# Autodesk Inventor assembly: main
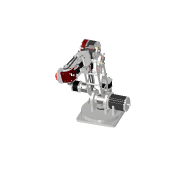
[picture p0: Inventor's stored thumbnail of the model, 180x180]
Saved by Autodesk Inventor 2020.3 (Build 243373000, 373)
## iProperties
Created: 2020-05-24
Part Number: main
Document SubType Name: Assembly
Designer: Svend
Author: Svend
## Documents named in this file (5)
- C:\Users\Svend\OneDrive\Documents\GitHub\BeerMinder\3D-model\mainAssembly\main.iam
- C:\Users\Svend\OneDrive\Documents\GitHub\BeerMinder\3D-model\axis3\axis3.iam
- C:\Users\Svend\OneDrive\Documents\GitHub\BeerMinder\3D-model\Base (Axis 1)\gefreesd\AssemblyGefreesdBasev2.iam
- C:\Users\Svend\OneDrive\Documents\GitHub\BeerMinder\3D-model\axis5_6\axis5_6  compact.iam
- C:\Users\Svend\OneDrive\Documents\GitHub\BeerMinder\3D-model\ControlBox\swithces\Assembly - V-156-1C25 micro switch (Idle).iam
## Components (8 placed, 4 different names)
1. axis3:1 [sub-assembly] — Mate:3, Mate:4, Mate:12, Mate:13, Mate:17, Mate:20, Mate:21, Mate:22, Mate:23, Mate:24, Mate:25, Mate:26, Mate:27
2. AssemblyGefreesdBasev2:1 [sub-assembly] — Mate:1, Mate:2, Flush:1, Mate:3, Mate:4, Mate:9, Mate:10, Angle:2, Flush:3
3. axis5_6  compact:1 [sub-assembly] — Mate:12, Mate:13
4. Assembly - V-156-1C25 micro switch (Idle):2 [sub-assembly]
5. Assembly - V-156-1C25 micro switch (Idle):1 [sub-assembly] — Mate:9, Mate:10, Angle:2, Flush:3
6. Assembly - V-156-1C25 micro switch (Idle):3 [sub-assembly] — Mate:20, Mate:21, Mate:22
7. Assembly - V-156-1C25 micro switch (Idle):4 [sub-assembly] — Mate:17, Mate:23, Mate:24
8. Assembly - V-156-1C25 micro switch (Idle):6 [sub-assembly] — Mate:25, Mate:26, Mate:27
## Relationships (23: Mate 18, Flush 3, Angle 2)
- Mate:1: AssemblyGefreesdBasev2:1
- Mate:2: AssemblyGefreesdBasev2:1
- Flush:1: AssemblyGefreesdBasev2:1
- Mate:3: axis3:1 ↔ AssemblyGefreesdBasev2:1
- Mate:4: axis3:1 ↔ AssemblyGefreesdBasev2:1
- [Mate] (2 mm): AssemblyGefreesdBasev2:1 ↔ Assembly - V-156-1C25 micro switch (Idle):2
- [Angle] (180 deg): AssemblyGefreesdBasev2:1 ↔ Assembly - V-156-1C25 micro switch (Idle):2
- [Flush] (19 mm): AssemblyGefreesdBasev2:1 ↔ Assembly - V-156-1C25 micro switch (Idle):2
- Mate:9 (95 mm): AssemblyGefreesdBasev2:1 ↔ Assembly - V-156-1C25 micro switch (Idle):1
- Mate:10: AssemblyGefreesdBasev2:1 ↔ Assembly - V-156-1C25 micro switch (Idle):1
- Angle:2 (0 deg): AssemblyGefreesdBasev2:1 ↔ Assembly - V-156-1C25 micro switch (Idle):1
- Flush:3 (35 mm): AssemblyGefreesdBasev2:1 ↔ Assembly - V-156-1C25 micro switch (Idle):1
- Mate:12: axis3:1 ↔ axis5_6  compact:1
- Mate:13: axis3:1 ↔ axis5_6  compact:1
- Mate:17: axis3:1 ↔ Assembly - V-156-1C25 micro switch (Idle):4
- Mate:20: axis3:1 ↔ Assembly - V-156-1C25 micro switch (Idle):3
- Mate:21: axis3:1 ↔ Assembly - V-156-1C25 micro switch (Idle):3
- Mate:22: axis3:1 ↔ Assembly - V-156-1C25 micro switch (Idle):3
- Mate:23: axis3:1 ↔ Assembly - V-156-1C25 micro switch (Idle):4
- Mate:24: axis3:1 ↔ Assembly - V-156-1C25 micro switch (Idle):4
- Mate:25: axis3:1 ↔ Assembly - V-156-1C25 micro switch (Idle):6
- Mate:26: axis3:1 ↔ Assembly - V-156-1C25 micro switch (Idle):6
- Mate:27: axis3:1 ↔ Assembly - V-156-1C25 micro switch (Idle):6
